# Autodesk Inventor assembly: EnsamblajeDodecaedro_V2
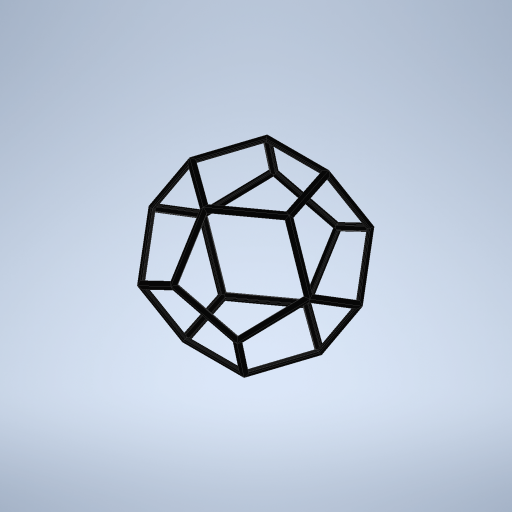
[picture p0: Inventor's stored thumbnail of the model, 512x512]
Saved by Autodesk Inventor 2024 (Build 280153000, 153)
## iProperties
Created: 2023-07-29
Part Number: EnsamblajeDodecaedro_V2
Document SubType Name: Assembly
Designer: sergi
Author: sergi
## Documents named in this file (2)
- C:\Users\sergi\OneDrive\Escritorio\Piso\Dodecaedro\EnsamblajeDodecaedro_V2.iam
- C:\Users\sergi\OneDrive\Escritorio\Piso\Dodecaedro\Perfil_V2.ipt
## Components (30 placed, 1 different names)
1. Perfil_V2:1 — Coincidencia:4, Coincidencia:5, Coincidencia:6
2. Perfil_V2:2 — Coincidencia:1, Coincidencia:2, Coincidencia:3, Coincidencia:4, Coincidencia:6, Coincidencia:23
3. Perfil_V2:3 — Coincidencia:1, Coincidencia:2, Coincidencia:3, Coincidencia:5, Coincidencia:13, Coincidencia:14, Coincidencia:48, Coincidencia:49, Coincidencia:50
4. Perfil_V2:4 — Coincidencia:13, Coincidencia:14
5. Perfil_V2:5 — Coincidencia:21, Coincidencia:22, Coincidencia:30, Coincidencia:31, Coincidencia:32
6. Perfil_V2:6 — Coincidencia:39, Coincidencia:40, Coincidencia:41
7. Perfil_V2:8 — Coincidencia:21, Coincidencia:22, Coincidencia:23
8. Perfil_V2:9 — Coincidencia:30, Coincidencia:31, Coincidencia:32
9. Perfil_V2:10 — Coincidencia:102, Coincidencia:103
10. Perfil_V2:11
11. Perfil_V2:12 — Coincidencia:39, Coincidencia:40, Coincidencia:41
12. Perfil_V2:14 — Coincidencia:68, Coincidencia:93, Coincidencia:94
13. Perfil_V2:15 — Coincidencia:48, Coincidencia:49, Coincidencia:50
14. Perfil_V2:16 — Coincidencia:57, Coincidencia:58, Coincidencia:59, Coincidencia:66
15. Perfil_V2:18 — Coincidencia:57, Coincidencia:58, Coincidencia:59, Coincidencia:67
16. Perfil_V2:19 — Coincidencia:75, Coincidencia:76, Coincidencia:77, Coincidencia:84, Coincidencia:85, Coincidencia:86
17. Perfil_V2:20 — Coincidencia:66, Coincidencia:67
18. Perfil_V2:21 — Coincidencia:68, Coincidencia:95
19. Perfil_V2:22 — Coincidencia:75, Coincidencia:76, Coincidencia:77
20. Perfil_V2:23
21. Perfil_V2:24
22. Perfil_V2:25 — Coincidencia:84, Coincidencia:85, Coincidencia:86
23. Perfil_V2:26
24. Perfil_V2:27 — Coincidencia:105
25. Perfil_V2:28
26. Perfil_V2:30 — Coincidencia:93, Coincidencia:94, Coincidencia:95
27. Perfil_V2:31 — Coincidencia:104, Coincidencia:106
28. Perfil_V2:32 — Coincidencia:102, Coincidencia:103
29. Perfil_V2:33
30. Perfil_V2:34 — Coincidencia:104, Coincidencia:105, Coincidencia:106
## Relationships (80: Mate 80)
- Coincidencia:1 [Mate]: Perfil_V2:2 ↔ Perfil_V2:3
- Coincidencia:2 [Mate]: Perfil_V2:2 ↔ Perfil_V2:3
- Coincidencia:3 [Mate]: Perfil_V2:2 ↔ Perfil_V2:3
- Coincidencia:4 [Mate]: Perfil_V2:1 ↔ Perfil_V2:2
- Coincidencia:5 [Mate]: Perfil_V2:1 ↔ Perfil_V2:3
- Coincidencia:6 [Mate]: Perfil_V2:1 ↔ Perfil_V2:2
- [Mate]: Perfil_V2:5 ↔ Perfil_V2:6
- [Mate]: Perfil_V2:5 ↔ Perfil_V2:6
- [Mate]: Perfil_V2:5 ↔ Perfil_V2:6
- [Mate]: Perfil_V2:4 ↔ Perfil_V2:5
- [Mate]: Perfil_V2:4 ↔ Perfil_V2:6
- [Mate]: Perfil_V2:4 ↔ Perfil_V2:5
- Coincidencia:13 [Mate]: Perfil_V2:3 ↔ Perfil_V2:4
- Coincidencia:14 [Mate]: Perfil_V2:3 ↔ Perfil_V2:4
- Coincidencia:21 [Mate]: Perfil_V2:5 ↔ Perfil_V2:8
- Coincidencia:22 [Mate]: Perfil_V2:5 ↔ Perfil_V2:8
- Coincidencia:23 [Mate]: Perfil_V2:2 ↔ Perfil_V2:8
- [Mate]: Perfil_V2:10 ↔ Perfil_V2:11
- [Mate]: Perfil_V2:10 ↔ Perfil_V2:11
- [Mate]: Perfil_V2:10 ↔ Perfil_V2:11
- [Mate]: Perfil_V2:9 ↔ Perfil_V2:10
- [Mate]: Perfil_V2:9 ↔ Perfil_V2:11
- [Mate]: Perfil_V2:9 ↔ Perfil_V2:10
- Coincidencia:30 [Mate]: Perfil_V2:5 ↔ Perfil_V2:9
- Coincidencia:31 [Mate]: Perfil_V2:5 ↔ Perfil_V2:9
- Coincidencia:32 [Mate]: Perfil_V2:5 ↔ Perfil_V2:9
- [Mate]: Perfil_V2:12 ↔ Perfil_V2:14
- Coincidencia:39 [Mate]: Perfil_V2:6 ↔ Perfil_V2:12
- Coincidencia:40 [Mate]: Perfil_V2:6 ↔ Perfil_V2:12
- Coincidencia:41 [Mate]: Perfil_V2:6 ↔ Perfil_V2:12
- [Mate]: Perfil_V2:15 ↔ Perfil_V2:16
- [Mate]: Perfil_V2:15 ↔ Perfil_V2:16
- Coincidencia:48 [Mate]: Perfil_V2:3 ↔ Perfil_V2:15
- Coincidencia:49 [Mate]: Perfil_V2:3 ↔ Perfil_V2:15
- Coincidencia:50 [Mate]: Perfil_V2:3 ↔ Perfil_V2:15
- Coincidencia:57 [Mate]: Perfil_V2:16 ↔ Perfil_V2:18
- Coincidencia:58 [Mate]: Perfil_V2:16 ↔ Perfil_V2:18
- Coincidencia:59 [Mate]: Perfil_V2:16 ↔ Perfil_V2:18
- [Mate]: Perfil_V2:20 ↔ Perfil_V2:21
- [Mate]: Perfil_V2:20 ↔ Perfil_V2:21
- [Mate]: Perfil_V2:20 ↔ Perfil_V2:21
- [Mate]: Perfil_V2:19 ↔ Perfil_V2:20
- [Mate]: Perfil_V2:19 ↔ Perfil_V2:21
- [Mate]: Perfil_V2:19 ↔ Perfil_V2:20
- Coincidencia:66 [Mate]: Perfil_V2:16 ↔ Perfil_V2:20
- Coincidencia:67 [Mate]: Perfil_V2:18 ↔ Perfil_V2:20
- Coincidencia:68 [Mate]: Perfil_V2:14 ↔ Perfil_V2:21
- [Mate]: Perfil_V2:23 ↔ Perfil_V2:24
- [Mate]: Perfil_V2:23 ↔ Perfil_V2:24
- [Mate]: Perfil_V2:23 ↔ Perfil_V2:24
- [Mate]: Perfil_V2:22 ↔ Perfil_V2:23
- [Mate]: Perfil_V2:22 ↔ Perfil_V2:24
- [Mate]: Perfil_V2:22 ↔ Perfil_V2:23
- Coincidencia:75 [Mate]: Perfil_V2:19 ↔ Perfil_V2:22
- Coincidencia:76 [Mate]: Perfil_V2:19 ↔ Perfil_V2:22
- Coincidencia:77 [Mate]: Perfil_V2:19 ↔ Perfil_V2:22
- [Mate]: Perfil_V2:26 ↔ Perfil_V2:27
- [Mate]: Perfil_V2:26 ↔ Perfil_V2:27
- [Mate]: Perfil_V2:26 ↔ Perfil_V2:27
- [Mate]: Perfil_V2:25 ↔ Perfil_V2:26
- [Mate]: Perfil_V2:25 ↔ Perfil_V2:27
- [Mate]: Perfil_V2:25 ↔ Perfil_V2:26
- Coincidencia:84 [Mate]: Perfil_V2:19 ↔ Perfil_V2:25
- Coincidencia:85 [Mate]: Perfil_V2:19 ↔ Perfil_V2:25
- Coincidencia:86 [Mate]: Perfil_V2:19 ↔ Perfil_V2:25
- [Mate]: Perfil_V2:28 ↔ Perfil_V2:30
- Coincidencia:93 [Mate]: Perfil_V2:14 ↔ Perfil_V2:30
- Coincidencia:94 [Mate]: Perfil_V2:14 ↔ Perfil_V2:30
- Coincidencia:95 [Mate]: Perfil_V2:21 ↔ Perfil_V2:30
- [Mate]: Perfil_V2:32 ↔ Perfil_V2:33
- [Mate]: Perfil_V2:32 ↔ Perfil_V2:33
- [Mate]: Perfil_V2:32 ↔ Perfil_V2:33
- [Mate]: Perfil_V2:31 ↔ Perfil_V2:32
- [Mate]: Perfil_V2:31 ↔ Perfil_V2:33
- [Mate]: Perfil_V2:31 ↔ Perfil_V2:32
- Coincidencia:102 [Mate]: Perfil_V2:10 ↔ Perfil_V2:32
- Coincidencia:103 [Mate]: Perfil_V2:10 ↔ Perfil_V2:32
- Coincidencia:104 [Mate]: Perfil_V2:31 ↔ Perfil_V2:34
- Coincidencia:105 [Mate]: Perfil_V2:27 ↔ Perfil_V2:34
- Coincidencia:106 [Mate]: Perfil_V2:31 ↔ Perfil_V2:34
## Named parameters: d6_d0 = 0 mm, d7_d1 = 0 mm, d8_d2 = 0 mm, d9_d3 = 0 mm, d10_d4 = 0 mm, d11_d5 = 0 mm, d23_d0 = 0 mm, d24_d1 = 0 mm, d25_d2 = 0 mm, d26_d3 = 0 mm, d27_d4 = 0 mm, d28_d5 = 0 mm, d36_d4 = 0 mm, d44_d3 = 0 mm, d46_d5 = 0 mm, d59_d0 = 0 mm, d60_d1 = 0 mm, d61_d2 = 0 mm, d62_d3 = 0 mm, d63_d4 = 0 mm, d64_d5 = 0 mm, d68_d0 = 0 mm, d69_d1 = 0 mm, d70_d2 = 0 mm, d71_d3 = 0 mm, d72_d4 = 0 mm, d73_d5 = 0 mm, d77_d0 = 0 mm, d78_d1 = 0 mm, d79_d2 = 0 mm, d80_d3 = 0 mm, d81_d4 = 0 mm, d82_d5 = 0 mm, d90_d4 = 0 mm, d95_d0 = 0 mm, d96_d1 = 0 mm, d97_d2 = 0 mm, d98_d3 = 0 mm, d99_d4 = 0 mm, d100_d5 = 0 mm
